# Autodesk Inventor assembly: DriverMount
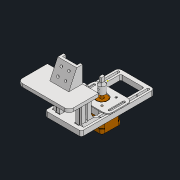
[picture p0: Inventor's stored thumbnail of the model, 180x180]
Saved by Autodesk Inventor 2022 (Build 260153000, 153)
## iProperties
Created: 2021-12-03
Part Number: DriverMount
Document SubType Name: Assembly
Designer: alber
Author: alber
## Documents named in this file (6)
- G:\My Drive\SPIN TEST Capstone\SpinTest_Capstone_Models\DriverMount.iam
- G:\My Drive\SPIN TEST Capstone\SpinTest_Capstone_Models\Driver_lock.ipt
- G:\My Drive\SPIN TEST Capstone\SpinTest_Capstone_Models\nema17.ipt
- G:\My Drive\SPIN TEST Capstone\SpinTest_Capstone_Models\sliderr.ipt
- G:\My Drive\SPIN TEST Capstone\SpinTest_Capstone_Models\VSlider.ipt
- G:\My Drive\SPIN TEST Capstone\SpinTest_Capstone_Models\Motor-Driver Coupler.ipt
## Components (5 placed, 5 different names)
1. Driver_lock:1 — Mate:4, Flush:2
2. nema17:1 — Cylindrical:1, Mate:7
3. NemaHolder — Flush:3, Mate:5, Cylindrical:1, Mate:7
4. Slider — Mate:4, Flush:2, Flush:3, Mate:5
5. Motor-Driver Coupler:1
## Relationships (6: Mate 3, Flush 2, CylindricalJoint 1)
- Mate:4 (1 mm): Driver_lock:1 ↔ Slider
- Flush:2 (-0.224 mm): Driver_lock:1 ↔ Slider
- Flush:3: NemaHolder ↔ Slider
- Mate:5: NemaHolder ↔ Slider
- Cylindrical:1: nema17:1 ↔ NemaHolder
- Mate:7: nema17:1 ↔ NemaHolder
